# Autodesk Inventor assembly: Body V7 Pi5 - Removable Electronics
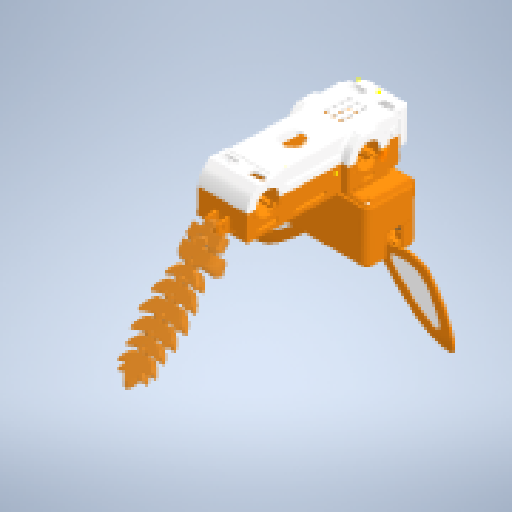
[picture p0: Inventor's stored thumbnail of the model, 512x512]
Saved by Autodesk Inventor 2024.2 (Build 282272000, 272)
## iProperties
Created: 2025-09-19
Part Number: Body V7 Pi5 - Removable Electronics
Document SubType Name: Assembly
Designer: AdminForWorker
Mass: 1197.51 g
Surface Area: 4986.69 cm^2
Volume: 827.285 cm^3
Density: 1.44752 g/cm^3
Title: Body V7 Pi5 - Removable Electronics v36
Author: AdminForWorker
## Documents named in this file (27)
- D:\dog\fox\construction\fox\body\тело лисы.iam
- D:\dog\fox\construction\fox\boards\3D_PCB4_2024-01-15 v3.iam
- D:\dog\fox\construction\fox\legs\Part222.ipt
- D:\dog\fox\construction\fox\body\верхняя часть.ipt
- D:\dog\fox\construction\fox\body\крышка камера.ipt
- D:\dog\fox\construction\fox\body\спина.ipt
- D:\dog\fox\construction\fox\body\шея.ipt
- D:\dog\fox\construction\fox\body\лицо.ipt
- D:\dog\fox\construction\fox\body\голова потолок.ipt
- D:\dog\fox\construction\fox\body\ухо правое.ipt
- D:\dog\fox\construction\fox\raspberry\0329_экран.ipt
- D:\dog\fox\construction\fox\body\JX Servo PDI-HV2006MG.ipt
- D:\dog\fox\construction\fox\body\накладка.ipt
- D:\dog\fox\construction\fox\boards\плата управления\плата управления.iam
- D:\dog\fox\construction\fox\boards\динамик\динамик.ipt
- D:\dog\fox\construction\fox\body\крепление сервоприводов.ipt
- D:\dog\fox\construction\fox\body\втавки в уши.ipt
- D:\dog\fox\construction\fox\body\крутилка3\крутилка3.ipt
- D:\dog\fox\construction\fox\raspberry\RPiAIHATPlusBoard\RPiAIHATPlusBoard.ipt
- D:\dog\fox\construction\fox\raspberry\RASPBERRY_PI_5\RASPBERRY_PI_5.ipt
- D:\dog\fox\construction\fox\body\упормоторов.ipt
- D:\dog\fox\construction\fox\body\низдляакума.ipt
- D:\dog\fox\construction\fox\body\подшипник.ipt
- D:\dog\fox\construction\fox\body\крепление ушей.ipt
- D:\dog\fox\construction\fox\body\носок.ipt
- D:\dog\fox\construction\fox\body\крепление ушей часть 2.ipt
- D:\alletz2\ETZ_10\construction\робот\GL60II\tail2.ipt
## Components (33 placed, 26 different names)
1. плата питания [sub-assembly] — Совмещение:3, Совмещение:4, Совмещение:5
2. крышка камера:1 — Совмещение:14, Совмещение:20, Заподлицо:69
3. основа тела — Заподлицо:1, Заподлицо:2, Заподлицо:3, Заподлицо:13, Заподлицо:42, Совмещение:25
4. верхняя часть:1 — Заподлицо:1, Заподлицо:2, Заподлицо:3, Совмещение:3, Совмещение:4, Совмещение:5, Заподлицо:14, Заподлицо:16, Заподлицо:17, Заподлицо:18, Совмещение:20, Заподлицо:40, Заподлицо:42, Совмещение:25, Совмещение:36, Заподлицо:69
5. потолок — Заподлицо:13, Заподлицо:14, Заподлицо:16, Заподлицо:17, Заподлицо:18, Заподлицо:19, Заподлицо:20, Заподлицо:43, Заподлицо:44
6. шея:1 — Заподлицо:19, Заподлицо:20, Заподлицо:43, Заподлицо:44, Заподлицо:45, Совмещение:37
7. лицо:1 — Заподлицо:24, Совмещение:6, Совмещение:7, Заподлицо:28, Совмещение:11, Совмещение:12, Совмещение:13, Заподлицо:29, С поворотом:5, Совмещение:23, Совмещение:24, Заподлицо:45, Совмещение:26, Совмещение:27, Заподлицо:49, Заподлицо:50, Совмещение:28, Заподлицо:67, Заподлицо:68, Совмещение:37
8. голова потолок:1 — Заподлицо:24, Совмещение:23, Совмещение:24
9. ухо правое:1 — Заподлицо:26, Заподлицо:38, Цилиндрический:1, Заподлицо:47, Заподлицо:52, Заподлицо:53, Совмещение:29, Заподлицо:54, Заподлицо:55, Заподлицо:56, Заподлицо:64
10. 0329_экран:1 — Совмещение:6, Совмещение:7, Заподлицо:28
11. JX Servo PDI-HV2006MG:1 — Совмещение:27, Совмещение:28, Заподлицо:51, Заподлицо:65, Заподлицо:66
12. JX Servo PDI-HV2006MG:2 — Совмещение:11, Совмещение:12, Совмещение:13, С поворотом:3
13. накладка:1 — Заподлицо:29
14. плата управления:1 [sub-assembly]
15. динамик:1 — Совмещение:14
16. крепление сервоприводов:1 — Совмещение:26
17. втавки в уши:1 — Заподлицо:38, Заподлицо:63
18. крутилка3:1 — С поворотом:3
19. крутилка3:2
20. RPiAIHATPlusBoard:1 — Совмещение:21, Совмещение:22
21. RASPBERRY_PI_5:1 — С поворотом:5, Совмещение:21, Совмещение:22
22. упормоторов:1 — Заподлицо:40
23. низдляакума:1
24. ухо правое:2 — Цилиндрический:2, Заподлицо:48, Совмещение:33, Заподлицо:63
25. подшипник:1 — Цилиндрический:1, Заподлицо:47
26. подшипник:2 — Цилиндрический:2, Заподлицо:48, Жесткий:1
27. крепление ушей:1 — Заподлицо:49, Заподлицо:50, Заподлицо:51, Заподлицо:52, Заподлицо:53, Совмещение:29, Заподлицо:57, Заподлицо:58, Заподлицо:65, Заподлицо:66, Заподлицо:67, Заподлицо:68
28. носок:1 — Заподлицо:54, Заподлицо:55, Заподлицо:56
29. крепление ушей часть 2:1 — Заподлицо:57, Заподлицо:58
30. крепление ушей часть 2:2
31. носок:2 — Жесткий:1, Совмещение:33
32. втавки в уши:2 — Заподлицо:64
33. tail2:1 — Совмещение:36
## Relationships (72: Flush 45, Mate 22, RevoluteJoint 2, CylindricalJoint 2, WeldJoint 1)
- Заподлицо:1 [Flush]: основа тела ↔ верхняя часть:1
- Заподлицо:2 [Flush]: основа тела ↔ верхняя часть:1
- Заподлицо:3 [Flush]: основа тела ↔ верхняя часть:1
- Совмещение:3 [Mate] (-15 mm): плата питания ↔ верхняя часть:1
- Совмещение:4 [Mate]: плата питания ↔ верхняя часть:1
- Совмещение:5 [Mate]: плата питания ↔ верхняя часть:1
- [Flush]: крышка камера:1 ↔ верхняя часть:1
- [Flush]: крышка камера:1 ↔ верхняя часть:1
- [Flush]: крышка камера:1 ↔ верхняя часть:1
- [Flush]: крышка камера:1 ↔ верхняя часть:1
- Заподлицо:13 [Flush]: основа тела ↔ потолок
- Заподлицо:14 [Flush]: верхняя часть:1 ↔ потолок
- Заподлицо:16 [Flush]: верхняя часть:1 ↔ потолок
- Заподлицо:17 [Flush]: верхняя часть:1 ↔ потолок
- Заподлицо:18 [Flush]: верхняя часть:1 ↔ потолок
- Заподлицо:19 [Flush]: потолок ↔ шея:1
- Заподлицо:20 [Flush]: потолок ↔ шея:1
- [Flush]: шея:1 ↔ лицо:1
- Заподлицо:24 [Flush]: лицо:1 ↔ голова потолок:1
- Заподлицо:26 [Flush]: ухо правое:1
- Совмещение:6 [Mate]: лицо:1 ↔ 0329_экран:1
- Совмещение:7 [Mate]: лицо:1 ↔ 0329_экран:1
- Заподлицо:28 [Flush]: лицо:1 ↔ 0329_экран:1
- Совмещение:11 [Mate] (-2 mm): лицо:1 ↔ JX Servo PDI-HV2006MG:2
- Совмещение:12 [Mate] (65 mm): лицо:1 ↔ JX Servo PDI-HV2006MG:2
- Совмещение:13 [Mate] (30 mm): лицо:1 ↔ JX Servo PDI-HV2006MG:2
- Заподлицо:29 [Flush]: лицо:1 ↔ накладка:1
- Совмещение:14 [Mate]: крышка камера:1 ↔ динамик:1
- Совмещение:20 [Mate]: крышка камера:1 ↔ верхняя часть:1
- Заподлицо:38 [Flush]: ухо правое:1 ↔ втавки в уши:1
- С поворотом:3 [RevoluteJoint]: JX Servo PDI-HV2006MG:2 ↔ крутилка3:1
- С поворотом:5 [RevoluteJoint]: лицо:1 ↔ RASPBERRY_PI_5:1
- Совмещение:21 [Mate] (1 mm): RPiAIHATPlusBoard:1 ↔ RASPBERRY_PI_5:1
- Совмещение:22 [Mate] (0.2 mm): RPiAIHATPlusBoard:1 ↔ RASPBERRY_PI_5:1
- Заподлицо:40 [Flush]: верхняя часть:1 ↔ упормоторов:1
- Совмещение:23 [Mate]: лицо:1 ↔ голова потолок:1
- Совмещение:24 [Mate]: лицо:1 ↔ голова потолок:1
- Заподлицо:42 [Flush]: основа тела ↔ верхняя часть:1
- Совмещение:25 [Mate]: основа тела ↔ верхняя часть:1
- Заподлицо:43 [Flush]: потолок ↔ шея:1
- Заподлицо:44 [Flush]: потолок ↔ шея:1
- Заподлицо:45 [Flush]: шея:1 ↔ лицо:1
- Совмещение:26 [Mate]: лицо:1 ↔ крепление сервоприводов:1
- [Flush]: основа тела ↔ низдляакума:1
- Цилиндрический:1 [CylindricalJoint]: ухо правое:1 ↔ подшипник:1
- Цилиндрический:2 [CylindricalJoint]: ухо правое:2 ↔ подшипник:2
- Совмещение:27 [Mate] (56 mm): лицо:1 ↔ JX Servo PDI-HV2006MG:1
- Заподлицо:47 [Flush]: ухо правое:1 ↔ подшипник:1
- Заподлицо:48 [Flush]: ухо правое:2 ↔ подшипник:2
- Заподлицо:49 [Flush]: лицо:1 ↔ крепление ушей:1
- Заподлицо:50 [Flush]: лицо:1 ↔ крепление ушей:1
- Совмещение:28 [Mate] (7 mm): лицо:1 ↔ JX Servo PDI-HV2006MG:1
- Заподлицо:51 [Flush] (20 mm): JX Servo PDI-HV2006MG:1 ↔ крепление ушей:1
- Заподлицо:52 [Flush]: ухо правое:1 ↔ крепление ушей:1
- Заподлицо:53 [Flush]: ухо правое:1 ↔ крепление ушей:1
- Совмещение:29 [Mate]: ухо правое:1 ↔ крепление ушей:1
- Заподлицо:54 [Flush]: ухо правое:1 ↔ носок:1
- Заподлицо:55 [Flush]: ухо правое:1 ↔ носок:1
- Заподлицо:56 [Flush]: ухо правое:1 ↔ носок:1
- Заподлицо:57 [Flush]: крепление ушей:1 ↔ крепление ушей часть 2:1
- Заподлицо:58 [Flush]: крепление ушей:1 ↔ крепление ушей часть 2:1
- Жесткий:1 [WeldJoint]: подшипник:2 ↔ носок:2
- Совмещение:33 [Mate]: ухо правое:2 ↔ носок:2
- Заподлицо:63 [Flush]: втавки в уши:1 ↔ ухо правое:2
- Заподлицо:64 [Flush]: ухо правое:1 ↔ втавки в уши:2
- Совмещение:36 [Mate]: верхняя часть:1 ↔ tail2:1
- Заподлицо:65 [Flush] (0.5 mm): JX Servo PDI-HV2006MG:1 ↔ крепление ушей:1
- Заподлицо:66 [Flush]: JX Servo PDI-HV2006MG:1 ↔ крепление ушей:1
- Заподлицо:67 [Flush]: лицо:1 ↔ крепление ушей:1
- Заподлицо:68 [Flush]: лицо:1 ↔ крепление ушей:1
- Заподлицо:69 [Flush]: крышка камера:1 ↔ верхняя часть:1
- Совмещение:37 [Mate]: шея:1 ↔ лицо:1
## Named parameters: d17_d6 = 0 mm, d106_d57 = 0 mm
